# Autodesk Inventor assembly: comb
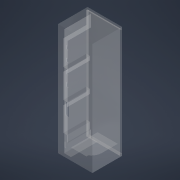
[picture p0: Inventor's stored thumbnail of the model, 180x180]
Saved by Autodesk Inventor 2022 (Build 260153000, 153)
## iProperties
Created: 2022-10-10
Part Number: comb
Document SubType Name: Assembly
Designer: 15628
Author: 15628
## Documents named in this file (3)
- C:\Users\15628\Desktop\CLOCK\comb.iam
- C:\Users\15628\Desktop\CLOCK\box.ipt
- C:\Users\15628\Desktop\CLOCK\top.ipt
## Components (2 placed, 2 different names)
1. box:1 — 表面齐平:1, 配合:1, 配合:2
2. top:1 — 表面齐平:1, 配合:1, 配合:2
## Relationships (3: Mate 2, Flush 1)
- 表面齐平:1 [Flush]: box:1 ↔ top:1
- 配合:1 [Mate]: box:1 ↔ top:1
- 配合:2 [Mate]: box:1 ↔ top:1
